# Autodesk Inventor assembly: Assembly1
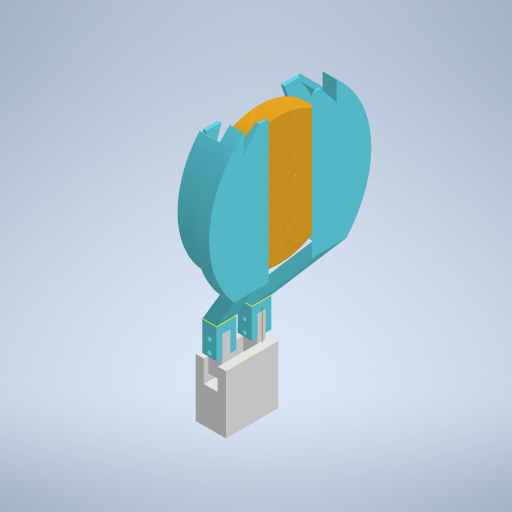
[picture p0: Inventor's stored thumbnail of the model, 512x512]
Saved by Autodesk Inventor 2024.3 (Build 283343000, 343)
## iProperties
Created: 2025-07-08
Part Number: Assembly1
Document SubType Name: Assembly
Designer: user
Author: user
## Documents named in this file (9)
- C:\Users\user\Desktop\Unal\Robotica\proyecto\garra neumatica\Assembly1.iam
- C:\Users\user\Desktop\Unal\Robotica\proyecto\garra neumatica\housing.ipt
- C:\Users\user\Desktop\Unal\Robotica\proyecto\garra neumatica\dedos.ipt
- C:\Users\user\Desktop\Unal\Robotica\proyecto\garra neumatica\eje.ipt
- C:\Users\user\Desktop\Unal\Robotica\proyecto\garra neumatica\eje_MIR.ipt
- C:\Users\user\Desktop\Unal\Robotica\proyecto\garra neumatica\dedos_MIR.ipt
- C:\Users\user\Desktop\Unal\Robotica\proyecto\garra neumatica\pinzatula1.ipt
- C:\Users\user\Desktop\Unal\Robotica\proyecto\garra neumatica\arepa.ipt
- C:\Users\user\Desktop\Unal\Robotica\proyecto\garra neumatica\pinzatula1_MIR.ipt
## Components (8 placed, 8 different names)
1. housing:1 — Flush:1, Rigid:1, Rotational:1, Mate:1, Angle:1, Rigid:2, Rotational:2, Mate:3, Angle:2
2. eje:1 — Flush:1, Rigid:1
3. dedos:1 — Rotational:1, Rigid:3
4. eje_MIR:1 — Rigid:2
5. dedos_MIR:1 — Rotational:2, Rigid:4
6. pinzatula1:1 — Rigid:3
7. arepa:1
8. pinzatula1_MIR:1 — Rigid:4
## Relationships (11: WeldJoint 4, RevoluteJoint 2, Mate 2, Angle 2, Flush 1)
- Flush:1: housing:1 ↔ eje:1
- Rigid:1 [WeldJoint]: housing:1 ↔ eje:1
- Rotational:1 [RevoluteJoint]: housing:1 ↔ dedos:1
- Mate:1: housing:1
- Angle:1 (0 deg): housing:1
- Rigid:2 [WeldJoint]: housing:1 ↔ eje_MIR:1
- Rotational:2 [RevoluteJoint]: housing:1 ↔ dedos_MIR:1
- Mate:3: housing:1
- Angle:2 (0 deg): housing:1
- Rigid:3 [WeldJoint]: dedos:1 ↔ pinzatula1:1
- Rigid:4 [WeldJoint]: dedos_MIR:1 ↔ pinzatula1_MIR:1
